# Autodesk Inventor assembly: BG_Rolle
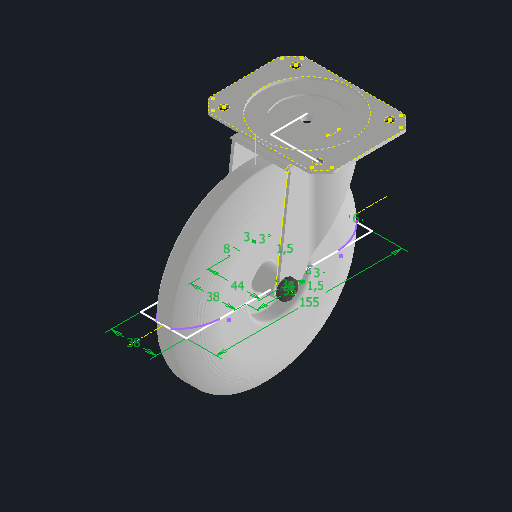
[picture p0: Inventor's stored thumbnail of the model, 512x512]
Saved by Autodesk Inventor 2026.3 (Build 303398000, 398)
## iProperties
Created: 2026-01-09
Part Number: BG_Rolle
Document SubType Name: Assembly
Designer: windows-desktop
Mass: 654.029 g
Surface Area: 995.24 cm^2
Volume: 630.234 cm^3
Density: 1.03775 g/cm^3
Author: windows-desktop
## Documents named in this file (7)
- C:\Users\bluhm\Desktop\Tretboot\Transport\BG_Rolle.iam
- C:\Users\bluhm\Desktop\Tretboot\Transport\Rolle.ipt
- C:\Users\bluhm\Desktop\Tretboot\Transport\RadBolzen.ipt
- C:\Users\bluhm\Desktop\Tretboot\Transport\Rolle_RippenStütze.ipt
- C:\Users\bluhm\Desktop\Tretboot\Transport\oberer_Rotierkörper_Rolle.ipt
- C:\Users\bluhm\Desktop\Tretboot\Normteile\ISO 7045(2)\DIN EN ISO 7045 - M8 x 20 - 4.8 - Z.ipt
- C:\Users\bluhm\Desktop\Tretboot\Normteile\ISO 7045(2)\DIN EN ISO 7045 - M8 x 16 - 4.8 - Z.ipt
## Components (6 placed, 6 different names)
1. Rolle:1 — Passend:2
2. RadBolzen:1 — Passend:1, Fluchtend:1, Fluchtend:2, Passend:2, Passend:3, Passend:4, Passend:5, Passend:6
3. Rolle_RippenStütze:1 — Passend:1, Fluchtend:1, Fluchtend:2, Einfügen:1
4. oberer_Rotierkörper_Rolle:1 — Einfügen:1
5. DIN EN ISO 7045 Z M8 x 20 - 4.8 - Z:1 — Passend:3, Passend:4
6. DIN EN ISO 7045 Z M8 x 16 - 4.8 - Z:1 — Passend:5, Passend:6
## Relationships (9: Mate 6, Flush 2, Insert 1)
- Passend:1 [Mate]: RadBolzen:1 ↔ Rolle_RippenStütze:1
- Fluchtend:1 [Flush]: RadBolzen:1 ↔ Rolle_RippenStütze:1
- Fluchtend:2 [Flush]: RadBolzen:1 ↔ Rolle_RippenStütze:1
- Passend:2 [Mate]: Rolle:1 ↔ RadBolzen:1
- Einfügen:1 [Insert]: Rolle_RippenStütze:1 ↔ oberer_Rotierkörper_Rolle:1
- Passend:3 [Mate]: RadBolzen:1 ↔ DIN EN ISO 7045 Z M8 x 20 - 4.8 - Z:1
- Passend:4 [Mate]: RadBolzen:1 ↔ DIN EN ISO 7045 Z M8 x 20 - 4.8 - Z:1
- Passend:5 [Mate]: RadBolzen:1 ↔ DIN EN ISO 7045 Z M8 x 16 - 4.8 - Z:1
- Passend:6 [Mate]: RadBolzen:1 ↔ DIN EN ISO 7045 Z M8 x 16 - 4.8 - Z:1
